# Autodesk Inventor assembly: assembly1
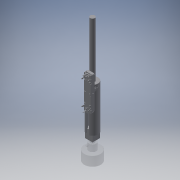
[picture p0: Inventor's stored thumbnail of the model, 180x180]
Saved by Autodesk Inventor 2018 (Build 220112000, 112)
## iProperties
Created: 2019-07-18
Part Number: assembly1
Document SubType Name: Assembly
Designer: aal_9
Author: aal_9
## Documents named in this file (6)
- C:\Users\aal_9\OneDrive\Documentos\Suiza\Courses\Tesis\CatheterLike\assembly1.iam
- C:\Users\aal_9\OneDrive\Documentos\Suiza\Courses\Tesis\CatheterLike\Handle.ipt
- C:\Users\aal_9\OneDrive\Documentos\Suiza\Courses\Tesis\CatheterLike\PotSensor.ipt
- C:\Users\aal_9\OneDrive\Documentos\Suiza\Courses\Tesis\CatheterLike\Rotation.ipt
- C:\Users\aal_9\OneDrive\Documentos\Suiza\Courses\Tesis\CatheterLike\PotHandle.ipt
- C:\Users\aal_9\OneDrive\Documentos\Suiza\Courses\Tesis\CatheterLike\PTA3043.ipt
## Components (5 placed, 5 different names)
1. Handle:1 — Mate:1, Mate:4, Mate:8, Mate:10, Flush:1
2. PotSensor:1 — Mate:2, Mate:3
3. Rotation:1 — Mate:1, Mate:4, Mate:5, Mate:6, Mate:7, Mate:9
4. PotHandle:1 — Mate:2, Mate:3, Mate:5, Mate:6, Mate:7, Mate:8
5. PTA3043:1 — Angle:1, Angle:2, Mate:9, Mate:10, Flush:1
## Relationships (13: Mate 10, Angle 2, Flush 1)
- Mate:1: Handle:1 ↔ Rotation:1
- Mate:2: PotSensor:1 ↔ PotHandle:1
- Mate:3: PotSensor:1 ↔ PotHandle:1
- Mate:4: Handle:1 ↔ Rotation:1
- Mate:5: Rotation:1 ↔ PotHandle:1
- Mate:6: Rotation:1 ↔ PotHandle:1
- Mate:7: Rotation:1 ↔ PotHandle:1
- Mate:8 (15 mm): Handle:1 ↔ PotHandle:1
- Angle:1 (180 deg): PTA3043:1
- Angle:2 (0 deg): PTA3043:1
- Mate:9: Rotation:1 ↔ PTA3043:1
- Mate:10 (-2 mm): Handle:1 ↔ PTA3043:1
- Flush:1 (-8 mm): Handle:1 ↔ PTA3043:1
